# Autodesk Inventor assembly: outer_MIR
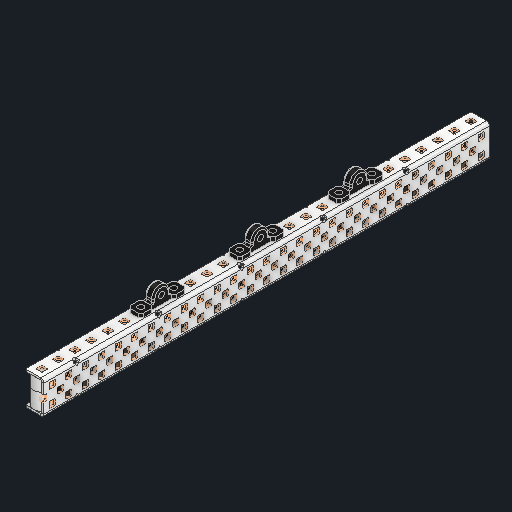
[picture p0: Inventor's stored thumbnail of the model, 512x512]
Saved by Autodesk Inventor 2024 (Build 280153000, 153)
## iProperties
Created: 2023-08-15
Part Number: outer_MIR
Document SubType Name: Assembly
Designer: avere
Author: avere
## Documents named in this file (10)
- D:\cad\scrap_v0.1\chassis\mirrored_parts\outer_MIR.iam
- D:\cad\scrap_v0.1\chassis\mirrored_parts\Alu C 1x2x1x27_MIR.ipt
- D:\cad\scrap_v0.1\chassis\mirrored_parts\Bearing Flat_MIR.ipt
- D:\cad\VEX-CAD-Inventor-1.41\Motion\Spacers\Spacer Nylon .500 OD\NSpacer White .500 OD x .375.ipt
- D:\cad\VEX-CAD-Inventor-1.41\Motion\Spacers\Spacer Nylon .500 OD\NSpacer White .500 OD x .500.ipt
- D:\cad\scrap_v0.1\chassis\mirrored_parts\LS Pillow Bearing Block_MIR.ipt
- D:\cad\VEX-CAD-Inventor-1.41\Structure\Standoff\Standoff .875.ipt
- D:\vex_robotics\hardware\cad\VEX-CAD-Inventor-1.41\Structure\Standoff.ipt
- D:\vex_robotics\hardware\cad\VEX-CAD-Inventor-1.41\Motion\Spacers\Spacer Nylon .500 OD.ipt
- D:\cad\VEX-CAD-Inventor-1.41\Motion\Shaft LS\Bearing Flat Low Profile.ipt
## Components (14 placed, 7 different names)
1. Alu C 1x2x1x27_MIR:1 — Mate:7, Insert:8, Mate:8, Insert:7, Insert:10, Insert:16, Insert:14, Insert:15, Insert:16, Insert:17, Insert:18, Mate:11, Mate:12, Mate:13, Mate:14, Mate:15, Insert:19, Insert:20, Insert:21, Mate:16, Mate:17, Mate:18
2. Bearing Flat_MIR:1 — Mate:7, Insert:8
3. Bearing Flat_MIR:2 — Mate:8, Insert:7
4. NSpacer White .500 OD x .375:1 — Insert:10, Insert:9
5. NSpacer White .500 OD x .500:2 — Insert:9
6. LS Pillow Bearing Block_MIR:1 — Insert:20, Mate:17
7. LS Pillow Bearing Block_MIR:2 — Insert:21, Mate:18
8. LS Pillow Bearing Block_MIR:3 — Insert:19, Mate:16
9. Standoff .875:1 — Insert:16
10. Bearing Flat Low Profile:1 — Insert:18, Mate:15
11. Bearing Flat Low Profile:6 — Insert:15, Mate:12
12. Bearing Flat Low Profile:7 — Insert:16, Mate:13
13. Bearing Flat Low Profile:10 — Insert:17, Mate:14
14. Bearing Flat Low Profile:11 — Insert:14, Mate:11
## Relationships (23: Insert 13, Mate 10)
- Mate:7: Alu C 1x2x1x27_MIR:1 ↔ Bearing Flat_MIR:1
- Insert:8: Alu C 1x2x1x27_MIR:1 ↔ Bearing Flat_MIR:1
- Mate:8: Alu C 1x2x1x27_MIR:1 ↔ Bearing Flat_MIR:2
- Insert:7: Alu C 1x2x1x27_MIR:1 ↔ Bearing Flat_MIR:2
- Insert:10: Alu C 1x2x1x27_MIR:1 ↔ NSpacer White .500 OD x .375:1
- Insert:9: NSpacer White .500 OD x .375:1 ↔ NSpacer White .500 OD x .500:2
- Insert:16: Alu C 1x2x1x27_MIR:1 ↔ Standoff .875:1
- Insert:14: Alu C 1x2x1x27_MIR:1 ↔ Bearing Flat Low Profile:11
- Insert:15: Alu C 1x2x1x27_MIR:1 ↔ Bearing Flat Low Profile:6
- Insert:16: Alu C 1x2x1x27_MIR:1 ↔ Bearing Flat Low Profile:7
- Insert:17: Alu C 1x2x1x27_MIR:1 ↔ Bearing Flat Low Profile:10
- Insert:18: Alu C 1x2x1x27_MIR:1 ↔ Bearing Flat Low Profile:1
- Mate:11: Alu C 1x2x1x27_MIR:1 ↔ Bearing Flat Low Profile:11
- Mate:12: Alu C 1x2x1x27_MIR:1 ↔ Bearing Flat Low Profile:6
- Mate:13: Alu C 1x2x1x27_MIR:1 ↔ Bearing Flat Low Profile:7
- Mate:14: Alu C 1x2x1x27_MIR:1 ↔ Bearing Flat Low Profile:10
- Mate:15: Alu C 1x2x1x27_MIR:1 ↔ Bearing Flat Low Profile:1
- Insert:19: Alu C 1x2x1x27_MIR:1 ↔ LS Pillow Bearing Block_MIR:3
- Insert:20: Alu C 1x2x1x27_MIR:1 ↔ LS Pillow Bearing Block_MIR:1
- Insert:21: Alu C 1x2x1x27_MIR:1 ↔ LS Pillow Bearing Block_MIR:2
- Mate:16: Alu C 1x2x1x27_MIR:1 ↔ LS Pillow Bearing Block_MIR:3
- Mate:17: Alu C 1x2x1x27_MIR:1 ↔ LS Pillow Bearing Block_MIR:1
- Mate:18: Alu C 1x2x1x27_MIR:1 ↔ LS Pillow Bearing Block_MIR:2
